# Autodesk Inventor assembly: screw
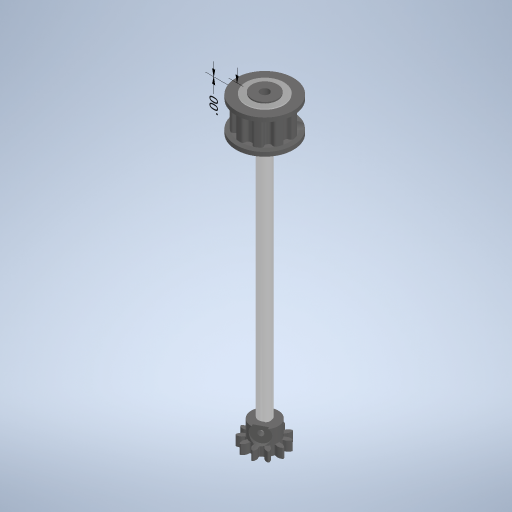
[picture p0: Inventor's stored thumbnail of the model, 512x512]
Saved by Autodesk Inventor 2024.1 (Build 281209000, 209)
## iProperties
Created: 2025-01-17
Part Number: screw
Document SubType Name: Assembly
Designer: hibik
Author: hibik
## Documents named in this file (7)
- C:\Users\hibik\Documents\Robomech\RESCUE\ORCA\hard\fork\fork\screw.iam
- C:\Users\hibik\Documents\Robomech\RESCUE\ORCA\hard\fork\fork\screw_screw.ipt
- C:\Users\hibik\Documents\Robomech\RESCUE\ORCA\hard\fork\fork\screw_gear_upper.ipt
- C:\Users\hibik\Documents\Robomech\RESCUE\ORCA\hard\std_parts\bearing_6_10_3.ipt
- C:\Users\hibik\Documents\Robomech\RESCUE\ORCA\hard\fork\fork\screw_bearing_setter.ipt
- C:\Users\hibik\Documents\Robomech\RESCUE\ORCA\hard\fork\fork\screw_gear_under_12.ipt
- C:\Users\hibik\Documents\Robomech\RESCUE\ORCA\hard\std_parts\bearing_3_6_2.5_noscrew.ipt
## Components (6 placed, 6 different names)
1. screw_screw:1 — 挿入:9, 挿入:11
2. bearing_6_10_3:1 — 挿入:7, 挿入:8
3. screw_bearing_setter:2 — 挿入:7, 挿入:9
4. bearing_3_6_2.5_noscrew:1 — 挿入:10, 挿入:11
5. screw_gear_under_12:1 — 挿入:10
6. screw_gear_upper:1 — 挿入:8
## Relationships (5: Insert 5)
- 挿入:7 [Insert]: bearing_6_10_3:1 ↔ screw_bearing_setter:2
- 挿入:8 [Insert]: bearing_6_10_3:1 ↔ screw_gear_upper:1
- 挿入:9 [Insert]: screw_screw:1 ↔ screw_bearing_setter:2
- 挿入:10 [Insert]: bearing_3_6_2.5_noscrew:1 ↔ screw_gear_under_12:1
- 挿入:11 [Insert] (1 mm): screw_screw:1 ↔ bearing_3_6_2.5_noscrew:1
